# Autodesk Inventor assembly: Shooter Assembly
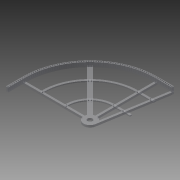
[picture p0: Inventor's stored thumbnail of the model, 180x180]
Saved by Autodesk Inventor 2013 (Build 170138000, 138)
## iProperties
Created: 2013-01-15
Part Number: Shooter Assembly
Document SubType Name: Assembly
Designer: actoennies
Author: actoennies
## Documents named in this file (4)
- H:\Robotics\Shooter\Shooter Assembly.iam
- \\NNHSSRV2.hs.sd203.org\ACToennies$\Robotics\Shooter\Bearing Mount v1.ipt
- \\NNHSSRV2.hs.sd203.org\ACToennies$\Robotics\Shooter\Runner Rails v1.ipt
- \\NNHSSRV2.hs.sd203.org\ACToennies$\Robotics\Shooter\Outer Rail v1.ipt
## Components (3 placed, 3 different names)
1. Bearing Mount v1:1 — Insert:1, Insert:2, Insert:3, Insert:4
2. Runner Rails v1:1 — Insert:1, Insert:2
3. Outer Rail v1:1 — Insert:3, Insert:4
## Relationships (4: Insert 4)
- Insert:1: Bearing Mount v1:1 ↔ Runner Rails v1:1
- Insert:2: Bearing Mount v1:1 ↔ Runner Rails v1:1
- Insert:3: Bearing Mount v1:1 ↔ Outer Rail v1:1
- Insert:4: Bearing Mount v1:1 ↔ Outer Rail v1:1
